# Autodesk Inventor assembly: test assy
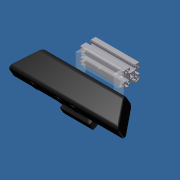
[picture p0: Inventor's stored thumbnail of the model, 180x180]
Saved by Autodesk Inventor 2012 (Build 160160000, 160)
## iProperties
Created: 2012-10-30
Part Number: test assy
Document SubType Name: Assembly
Designer: Ed
Author: Ed
## Documents named in this file (4)
- C:\Users\Ed\Documents\masters\CAD\Kinect\test assy.iam
- C:\Users\Ed\Documents\masters\CAD\Kinect\Kinect.ipt
- C:\Users\Ed\Documents\masters\CAD\Frame\aim rail cross brace.ipt
- C:\Users\Ed\Documents\masters\CAD\Kinect\kinect bracket.iam
## Components (3 placed, 3 different names)
1. Kinect:1 — Mate:3, Mate:4
2. aim rail cross brace:1 — Mate:1, Mate:2
3. kinect bracket:1 [sub-assembly] — Mate:1, Mate:2, Mate:3, Mate:4
## Relationships (4: Mate 4)
- Mate:1: aim rail cross brace:1 ↔ kinect bracket:1
- Mate:2: aim rail cross brace:1 ↔ kinect bracket:1
- Mate:3: Kinect:1 ↔ kinect bracket:1
- Mate:4: Kinect:1 ↔ kinect bracket:1
